# Autodesk Inventor assembly: arm_assembly
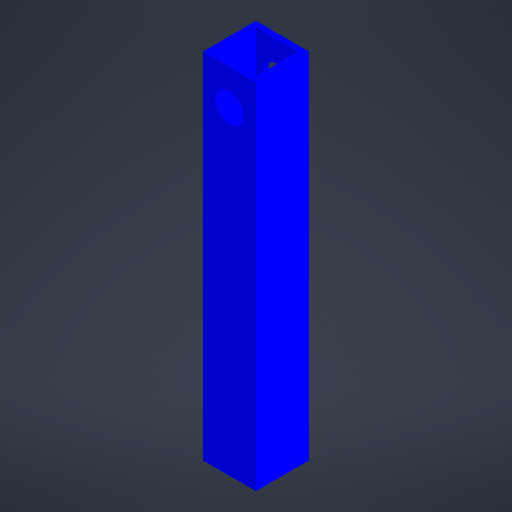
[picture p0: Inventor's stored thumbnail of the model, 512x512]
Saved by Autodesk Inventor 2024 (Build 280153000, 153)
## iProperties
Created: 2023-09-26
Part Number: arm_assembly
Document SubType Name: Assembly
Designer: user
Author: user
## Documents named in this file (2)
- D:\Docs\Robot\3d_v2\machine_body\arm_assembly.iam
- D:\Docs\Robot\3d_v2\base\arm.ipt
## Components (1 placed, 1 different names)
1. arm:1 — Совмещение:1, Совмещение:2, Совмещение:3
## Relationships (3: Mate 3)
- Совмещение:1 [Mate]: arm:1
- Совмещение:2 [Mate]: arm:1
- Совмещение:3 [Mate]: arm:1
